# Autodesk Inventor assembly: NP18-12
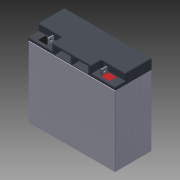
[picture p0: Inventor's stored thumbnail of the model, 180x180]
Saved by Autodesk Inventor 2018 (Build 220112000, 112)
## iProperties
Company: Autodesk Inc.
Category: Electrical
Created: 2017-12-13
Part Number: NP18-12
Document SubType Name: Assembly
Designer: Autodesk
Description: Battery, ,12 volt, 18 AH, Non-spillable
Catalog Web Link: https://www.enersys.com/default.aspx?langType=1033
Vendor: EnerSys
Author: Autodesk Inc.
Keywords: Separate Items
## Documents named in this file (3)
- D:\FIRST 2018\FIRST 2018 Inventor\FIRST 2018 Separate Items\NP18-12.iam
- D:\FIRST 2018\FIRST 2018 Inventor\FIRST 2018 Separate Items\Parts\Electrical_Yuasa_NP18-12_Top.ipt
- D:\FIRST 2018\FIRST 2018 Inventor\FIRST 2018 Separate Items\Parts\Electrical_Yuasa_Np18-12_Middle.ipt
## Components (2 placed, 2 different names)
1. Electrical_Yuasa_NP18-12_Top:1 — Flush:1
2. Electrical_Yuasa_Np18-12_Middle:1 — Flush:1
## Relationships (1: Flush 1)
- Flush:1: Electrical_Yuasa_NP18-12_Top:1 ↔ Electrical_Yuasa_Np18-12_Middle:1
